# Autodesk Inventor assembly: Assembly1
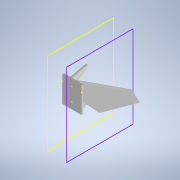
[picture p0: Inventor's stored thumbnail of the model, 180x180]
Saved by Autodesk Inventor 2020 (Build 240168000, 168)
## iProperties
Created: 2022-06-17
Part Number: Assembly1
Document SubType Name: Assembly
Designer: Steven
Author: Steven
## Documents named in this file (3)
- Y:\FPV drone stuff\0 Street League\Frames\dumb crap I shouldnt do\Assembly1.iam
- Y:\FPV drone stuff\0 Street League\Frames\dumb crap I shouldnt do\half fin mirror.ipt
- Y:\FPV drone stuff\0 Street League\Frames\PB-Kauri-X\3D prints\35 mm canopy\Tall KauriSpoilerFin.ipt
## Components (2 placed, 2 different names)
1. half fin mirror:1 — Mate:1, Flush:1, Flush:2
2. Tall KauriSpoilerFin:1 — Mate:1, Flush:1, Flush:2
## Relationships (3: Flush 2, Mate 1)
- Mate:1: half fin mirror:1 ↔ Tall KauriSpoilerFin:1
- Flush:1: half fin mirror:1 ↔ Tall KauriSpoilerFin:1
- Flush:2: half fin mirror:1 ↔ Tall KauriSpoilerFin:1
